# Autodesk Inventor assembly: Frezowanie_male No.3
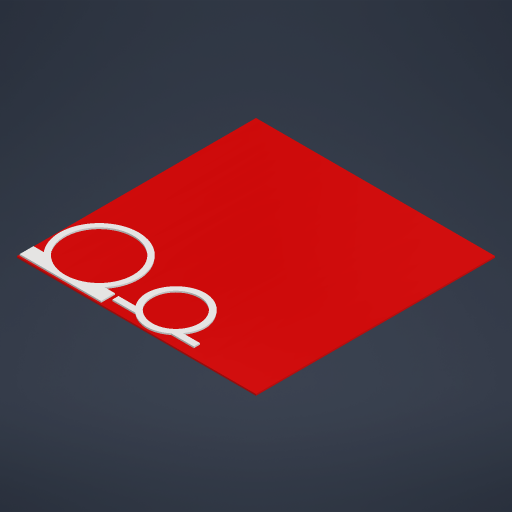
[picture p0: Inventor's stored thumbnail of the model, 512x512]
Saved by Autodesk Inventor 2023 (Build 270158000, 158)
## iProperties
Created: 2023-04-07
Part Number: Frezowanie_male No.3
Document SubType Name: Assembly
Designer: szykr
Author: szykr
## Documents named in this file (4)
- D:\Folder Instalacyjny\GitHub Pliki\Solaris\new model\Frez\Frezowanie_male No.3.iam
- D:\Folder Instalacyjny\GitHub Pliki\Solaris\new model\Frez\Laminat235x235.ipt
- D:\Folder Instalacyjny\GitHub Pliki\Solaris\new model\Frez\Troche Mniejsze(2-31)\Solid17.ipt
- D:\Folder Instalacyjny\GitHub Pliki\Solaris\new model\Frez\Troche Mniejsze(2-31)\Solid18.ipt
## Components (3 placed, 3 different names)
1. Laminat235x235:1 — Mate:1, Mate:2
2. Solid17:1 — Mate:1
3. Solid18:1 — Mate:2
## Relationships (2: Mate 2)
- Mate:1: Laminat235x235:1 ↔ Solid17:1
- Mate:2: Laminat235x235:1 ↔ Solid18:1
